# Autodesk Inventor assembly: Manipulator
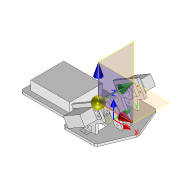
[picture p0: Inventor's stored thumbnail of the model, 180x180]
Saved by Autodesk Inventor 2020 (Build 240168000, 168)
## iProperties
Created: 2020-03-27
Part Number: Manipulator
Document SubType Name: Assembly
Designer: JakubTomaszewski
Mass: 263.816 g
Surface Area: 1015.48 cm^2
Volume: 305.917 cm^3
Density: 0.862378 g/cm^3
Author: JakubTomaszewski
## Documents named in this file (11)
- C:\Users\JakubTomaszewski\Documents\Inventor\Manipulator\Pierwsze Ogniwo.iam
- C:\Users\JakubTomaszewski\Documents\Inventor\Manipulator\Serwo.ipt
- C:\Users\JakubTomaszewski\Documents\Inventor\Manipulator\Serwo-końcówka.ipt
- C:\Users\JakubTomaszewski\Documents\Inventor\Manipulator\Podstawa_Gorna.ipt
- C:\Users\JakubTomaszewski\Documents\Inventor\Manipulator\Mocowanie_Serwa_1.ipt
- C:\Users\JakubTomaszewski\Documents\Inventor\Manipulator\Zawias-Serwo.ipt
- C:\Users\JakubTomaszewski\Documents\Inventor\Manipulator\Mocowanie_Serwa_2.ipt
- C:\Users\JakubTomaszewski\Documents\Inventor\Manipulator\Podtrzymanie_Osi.ipt
- C:\Users\JakubTomaszewski\Documents\Inventor\Manipulator\Zawias_Podtrzymanie_Osi.ipt
- C:\Users\JakubTomaszewski\Documents\Inventor\Manipulator\Oś.ipt
- C:\Users\JakubTomaszewski\Documents\Inventor\Manipulator\STM.ipt
## Components (15 placed, 10 different names)
1. Podstawa_Gorna:1 — Mocowanie_Serwa_1, Mocowanie_Serwa_2, Podtrzymanie_Osi_1, Podtrzymanie_Osi_2, Zawias_Podtrzymanie_Osi_1, Zawias_Podtrzymanie_Osi_2, przesuwne:1
2. Mocowanie_Serwa_1:1 — Mocowanie_Serwa_1, Zawias_Serwo_1, Serwo_1
3. Mocowanie_Serwa_2:1 — Serwo_2, Mocowanie_Serwa_2, Zawias_Serwo_2
4. Zawias-Serwo:1 — Zawias_Serwo_1
5. Zawias-Serwo:2 — Zawias_Serwo_2
6. Serwo:2 — Serwo_1, Końcówka_Serwo_1
7. Serwo:3 — Serwo_2, Końcówka_Serwo_2
8. Serwo-końcówka:2 — Końcówka_Serwo_1
9. Serwo-końcówka:3 — Oś, Końcówka_Serwo_2
10. Podtrzymanie_Osi:1 — Podtrzymanie_Osi_1
11. Podtrzymanie_Osi:2 — Podtrzymanie_Osi_2
12. Zawias_Podtrzymanie_Osi:1 — Zawias_Podtrzymanie_Osi_2
13. Zawias_Podtrzymanie_Osi:2 — Zawias_Podtrzymanie_Osi_1
14. Oś:1 — Oś
15. STM:1 — przesuwne:1
## Relationships (14: WeldJoint 10, RevoluteJoint 3, TranslationJoint 1)
- Mocowanie_Serwa_1 [WeldJoint]: Podstawa_Gorna:1 ↔ Mocowanie_Serwa_1:1
- Mocowanie_Serwa_2 [WeldJoint]: Podstawa_Gorna:1 ↔ Mocowanie_Serwa_2:1
- Zawias_Serwo_1 [WeldJoint]: Mocowanie_Serwa_1:1 ↔ Zawias-Serwo:1
- Zawias_Serwo_2 [WeldJoint]: Mocowanie_Serwa_2:1 ↔ Zawias-Serwo:2
- Serwo_1 [WeldJoint]: Mocowanie_Serwa_1:1 ↔ Serwo:2
- Serwo_2 [WeldJoint]: Mocowanie_Serwa_2:1 ↔ Serwo:3
- Końcówka_Serwo_1 [RevoluteJoint]: Serwo:2 ↔ Serwo-końcówka:2
- Końcówka_Serwo_2 [RevoluteJoint]: Serwo:3 ↔ Serwo-końcówka:3
- Podtrzymanie_Osi_1 [WeldJoint]: Podstawa_Gorna:1 ↔ Podtrzymanie_Osi:1
- Podtrzymanie_Osi_2 [WeldJoint]: Podstawa_Gorna:1 ↔ Podtrzymanie_Osi:2
- Zawias_Podtrzymanie_Osi_1 [WeldJoint]: Podstawa_Gorna:1 ↔ Zawias_Podtrzymanie_Osi:2
- Zawias_Podtrzymanie_Osi_2 [WeldJoint]: Podstawa_Gorna:1 ↔ Zawias_Podtrzymanie_Osi:1
- Oś [RevoluteJoint]: Serwo-końcówka:3 ↔ Oś:1
- przesuwne:1 [TranslationJoint]: Podstawa_Gorna:1 ↔ STM:1
